# Autodesk Inventor assembly: okragla mala napis
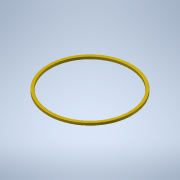
[picture p0: Inventor's stored thumbnail of the model, 180x180]
Saved by Autodesk Inventor 2021 (Build 250183000, 183)
## iProperties
Created: 2024-04-18
Part Number: okragla mala napis
Document SubType Name: Assembly
Designer: Michal
Author: Michal
## Documents named in this file (2)
- C:\Users\Michal\Documents\GitHub\PNW_PhotoBoothFrame_3D\okragla mala napis.iam
- C:\Users\Michal\Documents\GitHub\PNW_PhotoBoothFrame_3D\Kolo R600.ipt
## Components (1 placed, 1 different names)
1. Kolo R600:1 — Flush:26, Flush:27, Mate:35
## Relationships (3: Flush 2, Mate 1)
- Flush:26: Kolo R600:1
- Flush:27: Kolo R600:1
- Mate:35: Kolo R600:1
